# Autodesk Inventor assembly: Configuration 1
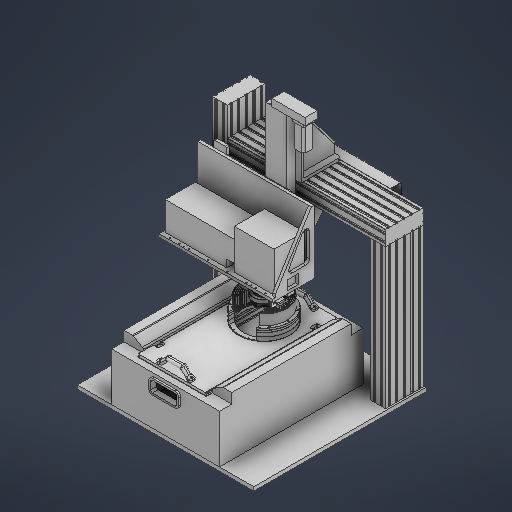
[picture p0: Inventor's stored thumbnail of the model, 512x512]
Saved by Autodesk Inventor 2025 (Build 290162000, 162)
## iProperties
Created: 2024-06-05
Part Number: Configuration 1
Document SubType Name: Assembly
Designer: AdminForWorker
Title: Printer Assembly v13
Author: AdminForWorker
## Documents named in this file (7)
- C:\Users\mayhe\OneDrive\Documents\GitHub\In-situ-monitoring-of-powder-bed-fusion-additive-manufacturing\system_development\Orichalcum\v0.2\Hardware_design\Full Printer Assembly\Printer Assembly.iam
- C:\Users\mayhe\OneDrive\Documents\GitHub\In-situ-monitoring-of-powder-bed-fusion-additive-manufacturing\system_development\Orichalcum\v0.2\Hardware_design\Full Printer Assembly\Laser w_ silver v4.iam
- C:\Users\mayhe\OneDrive\Documents\GitHub\In-situ-monitoring-of-powder-bed-fusion-additive-manufacturing\system_development\Orichalcum\v0.2\Hardware_design\Full Printer Assembly\Printer Body v6.ipt
- C:\Users\mayhe\OneDrive\Documents\GitHub\In-situ-monitoring-of-powder-bed-fusion-additive-manufacturing\system_development\Orichalcum\v0.2\Hardware_design\Full Printer Assembly\moving inner chamber piece v1 v2.ipt
- C:\Users\mayhe\OneDrive\Documents\GitHub\In-situ-monitoring-of-powder-bed-fusion-additive-manufacturing\system_development\Orichalcum\v0.2\Hardware_design\Full Printer Assembly\Printer Frame.ipt
- C:\Users\mayhe\OneDrive\Documents\GitHub\In-situ-monitoring-of-powder-bed-fusion-additive-manufacturing\system_development\Orichalcum\v0.2\Hardware_design\custom-cover\Custom Cover Full Assembly v0.2.iam
- C:\Users\mayhe\OneDrive\Documents\GitHub\In-situ-monitoring-of-powder-bed-fusion-additive-manufacturing\system_development\Orichalcum\v0.2\Hardware_design\galvo-scanner\Other Galvo\Non-ThorLabs Galvo.ipt
## Components (6 placed, 6 different names)
1. Laser w/ silver v4:1 [sub-assembly] — Mate:6
2. Printer Body v6:1 — Mate:1, Mate:2, Mate:3
3. moving inner chamber piece v1 v2:1
4. Part14
5. Custom Cover Full Assembly v0.2:1 [sub-assembly] — Mate:1, Mate:2, Mate:3
6. Non-ThorLabs Galvo:2 — Mate:6
## Relationships (4: Mate 4)
- Mate:1: Printer Body v6:1 ↔ Custom Cover Full Assembly v0.2:1
- Mate:2: Printer Body v6:1 ↔ Custom Cover Full Assembly v0.2:1
- Mate:3: Printer Body v6:1 ↔ Custom Cover Full Assembly v0.2:1
- Mate:6 (16 mm): Laser w/ silver v4:1 ↔ Non-ThorLabs Galvo:2
